# Autodesk Inventor assembly: Pakiet_zagrzany_gora
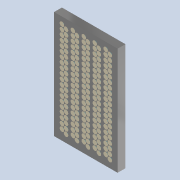
[picture p0: Inventor's stored thumbnail of the model, 180x180]
Saved by Autodesk Inventor 2021.3 (Build 253353000, 353)
## iProperties
Created: 2023-05-23
Part Number: Pakiet_zagrzany_gora
Document SubType Name: Assembly
Designer: User
Author: User
## Documents named in this file (6)
- E:\Inventor\Projekty\Modele Robotyzacja Procesów\Pakiet_zagrzany_gora.iam
- E:\Inventor\Projekty\Modele Robotyzacja Procesów\Model_Sita.ipt
- E:\Inventor\Projekty\Modele Robotyzacja Procesów\Model_Ogniwa.ipt
- E:\Inventor\Projekty\Modele Robotyzacja Procesów\tasiemka_do_zgrzewania_1.ipt
- tasiemka_do_zgrzewania_1.ipt
- E:\Inventor\Projekty\Modele Robotyzacja Procesów\tasiemka_do_zgrzewania_3.ipt
## Components (207 placed, 4 different names)
1. Model_Sita:1 — Zestawiające:1, Równoległe:1, Zestawiające:2, Równoległe:2, Równoległe:3, Równoległe:4, Równoległe:5, Równoległe:6
2. tasiemka_do_zgrzewania_1:1 — Zestawiające:4, Równoległe:4, Równoległe:6, Równoległe:8, Równoległe:9, Zestawiające:8
3. tasiemka_do_zgrzewania_1:2 — Zestawiające:3, Równoległe:3, Równoległe:5, Równoległe:7, Równoległe:10, Zestawiające:5
4. tasiemka_do_zgrzewania_3:1 — Równoległe:7, Zestawiające:5, Zestawiające:6, Zestawiające:12
5. tasiemka_do_zgrzewania_3:2 — Równoległe:10, Zestawiające:6, Zestawiające:7, Zestawiające:11
6. tasiemka_do_zgrzewania_3:3 — Równoległe:9, Zestawiające:7, Zestawiające:10
7. tasiemka_do_zgrzewania_3:4 — Równoległe:8, Zestawiające:8, Zestawiające:9
8. Model_Ogniwa:1 — Zestawiające:1, Równoległe:1
9. Model_Ogniwa:2
10. Model_Ogniwa:3
11. Model_Ogniwa:4
12. Model_Ogniwa:5
13. Model_Ogniwa:6
14. Model_Ogniwa:7
15. Model_Ogniwa:8
16. Model_Ogniwa:9
17. Model_Ogniwa:10
18. Model_Ogniwa:11
19. Model_Ogniwa:12
20. Model_Ogniwa:13
21. Model_Ogniwa:14
22. Model_Ogniwa:15
23. Model_Ogniwa:16
24. Model_Ogniwa:17
25. Model_Ogniwa:18
26. Model_Ogniwa:19
27. Model_Ogniwa:20 — Zestawiające:4
28. Model_Ogniwa:21
29. Model_Ogniwa:22
30. Model_Ogniwa:23
31. Model_Ogniwa:24
32. Model_Ogniwa:25
33. Model_Ogniwa:26
34. Model_Ogniwa:27
35. Model_Ogniwa:28
36. Model_Ogniwa:29
37. Model_Ogniwa:30
38. Model_Ogniwa:31
39. Model_Ogniwa:32
40. Model_Ogniwa:33
41. Model_Ogniwa:34
42. Model_Ogniwa:35
43. Model_Ogniwa:36
44. Model_Ogniwa:37
45. Model_Ogniwa:38
46. Model_Ogniwa:39
47. Model_Ogniwa:40
48. Model_Ogniwa:41
49. Model_Ogniwa:42
50. Model_Ogniwa:43
51. Model_Ogniwa:44
52. Model_Ogniwa:45
53. Model_Ogniwa:46
54. Model_Ogniwa:47
55. Model_Ogniwa:48
56. Model_Ogniwa:49
57. Model_Ogniwa:50
58. Model_Ogniwa:51
59. Model_Ogniwa:52
60. Model_Ogniwa:53
61. Model_Ogniwa:54
62. Model_Ogniwa:55
63. Model_Ogniwa:56
64. Model_Ogniwa:57
65. Model_Ogniwa:58
66. Model_Ogniwa:59
67. Model_Ogniwa:60
68. Model_Ogniwa:61
69. Model_Ogniwa:62
70. Model_Ogniwa:63
71. Model_Ogniwa:64
72. Model_Ogniwa:65
73. Model_Ogniwa:66
74. Model_Ogniwa:67
75. Model_Ogniwa:68
76. Model_Ogniwa:69
77. Model_Ogniwa:70
78. Model_Ogniwa:71
79. Model_Ogniwa:72
80. Model_Ogniwa:73
81. Model_Ogniwa:74
82. Model_Ogniwa:75
83. Model_Ogniwa:76
84. Model_Ogniwa:77
85. Model_Ogniwa:78
86. Model_Ogniwa:79 — Zestawiające:11
87. Model_Ogniwa:80
88. Model_Ogniwa:81
89. Model_Ogniwa:82
90. Model_Ogniwa:83
91. Model_Ogniwa:84
92. Model_Ogniwa:85
93. Model_Ogniwa:86
94. Model_Ogniwa:87
95. Model_Ogniwa:88
96. Model_Ogniwa:89
97. Model_Ogniwa:90
98. Model_Ogniwa:91
99. Model_Ogniwa:92
100. Model_Ogniwa:93
101. Model_Ogniwa:94
102. Model_Ogniwa:95
103. Model_Ogniwa:96
104. Model_Ogniwa:97
105. Model_Ogniwa:98
106. Model_Ogniwa:99 — Zestawiające:12
107. Model_Ogniwa:100
108. Model_Ogniwa:101 — Zestawiające:2, Równoległe:2
109. Model_Ogniwa:102
110. Model_Ogniwa:103
111. Model_Ogniwa:104
112. Model_Ogniwa:105
113. Model_Ogniwa:106
114. Model_Ogniwa:107
115. Model_Ogniwa:108
116. Model_Ogniwa:109
117. Model_Ogniwa:110
118. Model_Ogniwa:111
119. Model_Ogniwa:112
120. Model_Ogniwa:113
121. Model_Ogniwa:114
122. Model_Ogniwa:115
123. Model_Ogniwa:116
124. Model_Ogniwa:117
125. Model_Ogniwa:118
126. Model_Ogniwa:119
127. Model_Ogniwa:120 — Zestawiające:9
128. Model_Ogniwa:121
129. Model_Ogniwa:122
130. Model_Ogniwa:123
131. Model_Ogniwa:124
132. Model_Ogniwa:125
133. Model_Ogniwa:126
134. Model_Ogniwa:127
135. Model_Ogniwa:128
136. Model_Ogniwa:129
137. Model_Ogniwa:130
138. Model_Ogniwa:131
139. Model_Ogniwa:132
140. Model_Ogniwa:133
141. Model_Ogniwa:134
142. Model_Ogniwa:135
143. Model_Ogniwa:136
144. Model_Ogniwa:137
145. Model_Ogniwa:138
146. Model_Ogniwa:139 — Zestawiające:10
147. Model_Ogniwa:140
148. Model_Ogniwa:141
149. Model_Ogniwa:142
150. Model_Ogniwa:143
151. Model_Ogniwa:144
152. Model_Ogniwa:145
153. Model_Ogniwa:146
154. Model_Ogniwa:147
155. Model_Ogniwa:148
156. Model_Ogniwa:149
157. Model_Ogniwa:150
158. Model_Ogniwa:151
159. Model_Ogniwa:152
160. Model_Ogniwa:153
161. Model_Ogniwa:154
162. Model_Ogniwa:155
163. Model_Ogniwa:156
164. Model_Ogniwa:157
165. Model_Ogniwa:158
166. Model_Ogniwa:159
167. Model_Ogniwa:160
168. Model_Ogniwa:161
169. Model_Ogniwa:162
170. Model_Ogniwa:163
171. Model_Ogniwa:164
172. Model_Ogniwa:165
173. Model_Ogniwa:166
174. Model_Ogniwa:167
175. Model_Ogniwa:168
176. Model_Ogniwa:169
177. Model_Ogniwa:170
178. Model_Ogniwa:171
179. Model_Ogniwa:172
180. Model_Ogniwa:173
181. Model_Ogniwa:174
182. Model_Ogniwa:175
183. Model_Ogniwa:176
184. Model_Ogniwa:177
185. Model_Ogniwa:178
186. Model_Ogniwa:179
187. Model_Ogniwa:180
188. Model_Ogniwa:181
189. Model_Ogniwa:182
190. Model_Ogniwa:183
191. Model_Ogniwa:184
192. Model_Ogniwa:185
193. Model_Ogniwa:186
194. Model_Ogniwa:187
195. Model_Ogniwa:188
196. Model_Ogniwa:189
197. Model_Ogniwa:190
198. Model_Ogniwa:191
199. Model_Ogniwa:192
200. Model_Ogniwa:193
201. Model_Ogniwa:194
202. Model_Ogniwa:195
203. Model_Ogniwa:196
204. Model_Ogniwa:197
205. Model_Ogniwa:198
206. Model_Ogniwa:199
207. Model_Ogniwa:200 — Zestawiające:3
## Component patterns: (5 elements), (5 elements), (20 elements, first: Model_Ogniwa:1), Szyk komponentów 1:2 (20 elements), Szyk komponentów 1:3 (20 elements), Szyk komponentów 1:4 (20 elements), Szyk komponentów 1:5 (20 elements), (20 elements, first: Model_Ogniwa:101), Szyk komponentów 3:2 (20 elements), Szyk komponentów 3:3 (20 elements), Szyk komponentów 3:4 (20 elements), Szyk komponentów 3:5 (20 elements)
## Relationships (22: Mate 12, Flush 10)
- Zestawiające:1 [Mate]: Model_Sita:1 ↔ Model_Ogniwa:1
- Równoległe:1 [Flush]: Model_Sita:1 ↔ Model_Ogniwa:1
- Zestawiające:2 [Mate]: Model_Sita:1 ↔ Model_Ogniwa:101
- Równoległe:2 [Flush]: Model_Sita:1 ↔ Model_Ogniwa:101
- Zestawiające:3 [Mate]: tasiemka_do_zgrzewania_1:2 ↔ Model_Ogniwa:200
- Równoległe:3 [Flush] (54 mm): Model_Sita:1 ↔ tasiemka_do_zgrzewania_1:2
- Zestawiające:4 [Mate]: tasiemka_do_zgrzewania_1:1 ↔ Model_Ogniwa:20
- Równoległe:4 [Flush] (54 mm): Model_Sita:1 ↔ tasiemka_do_zgrzewania_1:1
- Równoległe:5 [Flush] (60 mm): Model_Sita:1 ↔ tasiemka_do_zgrzewania_1:2
- Równoległe:6 [Flush] (50 mm): Model_Sita:1 ↔ tasiemka_do_zgrzewania_1:1
- Równoległe:7 [Flush]: tasiemka_do_zgrzewania_1:2 ↔ tasiemka_do_zgrzewania_3:1
- Równoległe:8 [Flush]: tasiemka_do_zgrzewania_1:1 ↔ tasiemka_do_zgrzewania_3:4
- Równoległe:9 [Flush]: tasiemka_do_zgrzewania_1:1 ↔ tasiemka_do_zgrzewania_3:3
- Równoległe:10 [Flush]: tasiemka_do_zgrzewania_1:2 ↔ tasiemka_do_zgrzewania_3:2
- Zestawiające:5 [Mate] (10 mm): tasiemka_do_zgrzewania_1:2 ↔ tasiemka_do_zgrzewania_3:1
- Zestawiające:6 [Mate] (15 mm): tasiemka_do_zgrzewania_3:1 ↔ tasiemka_do_zgrzewania_3:2
- Zestawiające:7 [Mate] (20 mm): tasiemka_do_zgrzewania_3:2 ↔ tasiemka_do_zgrzewania_3:3
- Zestawiające:8 [Mate] (10 mm): tasiemka_do_zgrzewania_1:1 ↔ tasiemka_do_zgrzewania_3:4
- Zestawiające:9 [Mate]: tasiemka_do_zgrzewania_3:4 ↔ Model_Ogniwa:120
- Zestawiające:10 [Mate]: tasiemka_do_zgrzewania_3:3 ↔ Model_Ogniwa:139
- Zestawiające:11 [Mate]: tasiemka_do_zgrzewania_3:2 ↔ Model_Ogniwa:79
- Zestawiające:12 [Mate]: tasiemka_do_zgrzewania_3:1 ↔ Model_Ogniwa:99
